# Autodesk Inventor assembly: uchwyt silnika
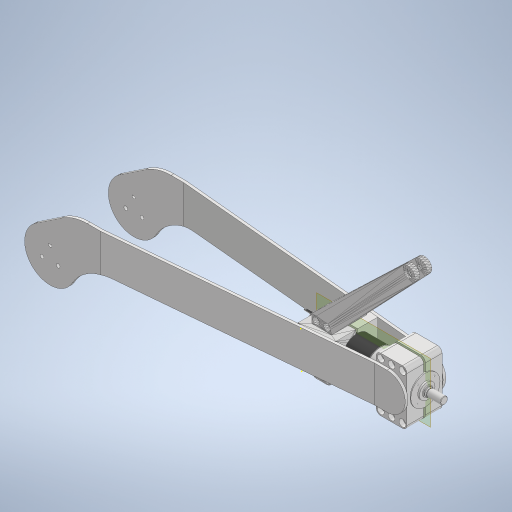
[picture p0: Inventor's stored thumbnail of the model, 512x512]
Saved by Autodesk Inventor 2023 (Build 270158000, 158)
## iProperties
Created: 2023-05-31
Part Number: uchwyt silnika
Document SubType Name: Assembly
Designer: Kamil
Author: Kamil
## Documents named in this file (7)
- C:\Users\Kamil\Desktop\KONARM_2\czlon 4\czlon4_zlozenie.iam
- C:\Users\Kamil\Desktop\KONARM_2\czlon 3\Faulhaber 3272G012C R.ipt
- C:\Users\Kamil\Desktop\KONARM_2\czlon 4\uchwyt_MIR.ipt
- C:\Users\Kamil\Desktop\KONARM_2\czlon 4\bok2_MIR.ipt
- C:\Users\Kamil\Desktop\KONARM_2\czlon 4\bok2_MIR_MIR.ipt
- C:\Users\Kamil\Desktop\KONARM_2\czlon 4\uchwyt_kopia.ipt
- C:\Users\Kamil\Desktop\uchwyt21.ipt
## Components (7 placed, 6 different names)
1. Faulhaber 3272G012C R:1 — Zestawiające:6
2. uchwyt_MIR:1 — Zestawiające:2, Równoległe:1, Równoległe:2
3. bok2_MIR:1 — Zestawiające:5
4. bok2_MIR_MIR:1 — Zestawiające:3, Zestawiające:4
5. uchwyt_kopia:1 — Zestawiające:4, Równoległe:3, Równoległe:4
6. uchwyt21:1 — Zestawiające:3, Równoległe:1, Równoległe:2
7. uchwyt_kopia:2 — Zestawiające:5, Zestawiające:6, Równoległe:3, Równoległe:4
## Relationships (9: Mate 5, Flush 4)
- Zestawiające:2 [Mate] (1 mm): uchwyt_MIR:1
- Zestawiające:3 [Mate]: bok2_MIR_MIR:1 ↔ uchwyt21:1
- Równoległe:1 [Flush]: uchwyt_MIR:1 ↔ uchwyt21:1
- Równoległe:2 [Flush]: uchwyt_MIR:1 ↔ uchwyt21:1
- Zestawiające:4 [Mate]: bok2_MIR_MIR:1 ↔ uchwyt_kopia:1
- Zestawiające:5 [Mate]: bok2_MIR:1 ↔ uchwyt_kopia:2
- Zestawiające:6 [Mate]: Faulhaber 3272G012C R:1 ↔ uchwyt_kopia:2
- Równoległe:3 [Flush]: uchwyt_kopia:1 ↔ uchwyt_kopia:2
- Równoległe:4 [Flush]: uchwyt_kopia:1 ↔ uchwyt_kopia:2
